# Autodesk Inventor assembly: assembly
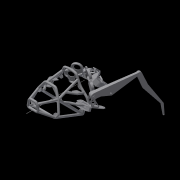
[picture p0: Inventor's stored thumbnail of the model, 180x180]
Saved by Autodesk Inventor 2020 (Build 240168000, 168)
## iProperties
Created: 2020-03-24
Part Number: assembly
Document SubType Name: Assembly
Designer: valer
Author: valer
## Documents named in this file (6)
- C:\Users\valer\Desktop\drummingrobot\src\Robot.iam
- C:\Users\valer\Desktop\drummingrobot\src\Chest.ipt
- C:\Users\valer\Desktop\drummingrobot\src\HeadScaled.ipt
- C:\Users\valer\Desktop\drummingrobot\src\UpperArmMount.ipt
- C:\Users\valer\Desktop\drummingrobot\src\UpperArmServoDynamixelXM430-W350-T.ipt
- C:\Users\valer\Desktop\drummingrobot\src\Arm.iam
## Components (6 placed, 5 different names)
1. Chest:1 — Angle:1, Mate:24, Mate:26, Mate:27
2. HeadScaled:1
3. UpperArmServoDynamixelXM430-W350-T:1 — Angle:1, Mate:28, Mate:33, Mate:34
4. UpperArmMount:2 — Mate:24, Mate:26, Mate:27, Mate:28, Mate:31, Mate:32, Mate:33, Mate:35, Mate:36
5. UpperArmMount:3 — Mate:31, Mate:32, Mate:34
6. Arm:1 [sub-assembly] — Mate:35, Mate:36
## Relationships (11: Mate 10, Angle 1)
- Angle:1 (0 deg): Chest:1 ↔ UpperArmServoDynamixelXM430-W350-T:1
- Mate:24 (12.7 mm): Chest:1 ↔ UpperArmMount:2
- Mate:26: Chest:1 ↔ UpperArmMount:2
- Mate:27: Chest:1 ↔ UpperArmMount:2
- Mate:28: UpperArmServoDynamixelXM430-W350-T:1 ↔ UpperArmMount:2
- Mate:31: UpperArmMount:2 ↔ UpperArmMount:3
- Mate:32: UpperArmMount:2 ↔ UpperArmMount:3
- Mate:33: UpperArmServoDynamixelXM430-W350-T:1 ↔ UpperArmMount:2
- Mate:34: UpperArmServoDynamixelXM430-W350-T:1 ↔ UpperArmMount:3
- Mate:35: UpperArmMount:2 ↔ Arm:1
- Mate:36: UpperArmMount:2 ↔ Arm:1
